# Autodesk Inventor assembly: DriveTrainPlateMecanum2017-18BackUp
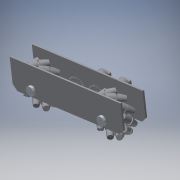
[picture p0: Inventor's stored thumbnail of the model, 180x180]
Saved by Autodesk Inventor 2017 (Build 210142000, 142)
## iProperties
Created: 2017-09-16
Part Number: DriveTrainPlateMecanum2017-18BackUp
Document SubType Name: Assembly
Designer: User
Author: User
## Documents named in this file (8)
- C:\Robotics\CAD\2017-18_CAD\DriveTrainMecanumDemo1.iam
- C:\Robotics\CAD\2017-18_CAD\MecanumDriveTrainPlate17-18.ipt
- C:\Robotics\CAD\2017-18_CAD\LeftDriveTrainMecanum2017-18.iam
- C:\Robotics\CAD\COTSParts\Motors\Andymark 2964  NeveRest 40 Motor.ipt
- C:\Robotics\CAD\2017-18_CAD\MecanumDriveTrainPlate17-18-NoMotor.ipt
- C:\Robotics\CAD\COTSParts\Tetrix\tetrix-motor-mounts-1.snapshot.1\Tetrex 2pc motor mount.ipt
- C:\Robotics\CAD\COTSParts\Actobotics\615 parts\615114.ipt
- C:\Robotics\CAD\COTSParts\Actobotics\545 parts\545576.ipt
## Components (12 placed, 7 different names)
1. LeftDriveTrainMecanum2017-18:1 [sub-assembly] — Mate:5, Mate:9, Mate:11, Mate:12
2. LeftDriveTrainMecanum2017-18:2 [sub-assembly] — Mate:6, Mate:7, Mate:10, Mate:13, Flush:3
3. MecanumDriveTrainPlate17-18:2 — Mate:5, Mate:6, Mate:7, Mate:9, Mate:12, Insert:1, Insert:2, Insert:3, Insert:4
4. Andymark 2964  NeveRest 40 Motor:1 — Mate:15, Flush:2, Mate:17
5. Andymark 2964  NeveRest 40 Motor:2 — Mate:14, Flush:1, Mate:16
6. MecanumDriveTrainPlate17-18-NoMotor:1 — Mate:10, Mate:11, Mate:13
7. Tetrex 2pc motor mount:1 — Insert:1, Insert:2, Mate:15, Flush:2
8. Tetrex 2pc motor mount:2 — Insert:3, Insert:4, Mate:14, Flush:1
9. 615114:1 — Mate:16, Flush:3, Flush:4, Insert:7, Insert:8
10. 615114:2 — Mate:17, Flush:4, Insert:5, Insert:6
11. 545576:1 — Insert:7, Insert:8
12. 545576:2 — Insert:5, Insert:6
## Relationships (24: Mate 12, Insert 8, Flush 4)
- Mate:5: LeftDriveTrainMecanum2017-18:1 ↔ MecanumDriveTrainPlate17-18:2
- Mate:6: LeftDriveTrainMecanum2017-18:2 ↔ MecanumDriveTrainPlate17-18:2
- Mate:7: LeftDriveTrainMecanum2017-18:2 ↔ MecanumDriveTrainPlate17-18:2
- Mate:9: LeftDriveTrainMecanum2017-18:1 ↔ MecanumDriveTrainPlate17-18:2
- Mate:10: LeftDriveTrainMecanum2017-18:2 ↔ MecanumDriveTrainPlate17-18-NoMotor:1
- Mate:11: LeftDriveTrainMecanum2017-18:1 ↔ MecanumDriveTrainPlate17-18-NoMotor:1
- Mate:12: LeftDriveTrainMecanum2017-18:1 ↔ MecanumDriveTrainPlate17-18:2
- Mate:13: LeftDriveTrainMecanum2017-18:2 ↔ MecanumDriveTrainPlate17-18-NoMotor:1
- Insert:1: MecanumDriveTrainPlate17-18:2 ↔ Tetrex 2pc motor mount:1
- Insert:2: MecanumDriveTrainPlate17-18:2 ↔ Tetrex 2pc motor mount:1
- Insert:3: MecanumDriveTrainPlate17-18:2 ↔ Tetrex 2pc motor mount:2
- Insert:4: MecanumDriveTrainPlate17-18:2 ↔ Tetrex 2pc motor mount:2
- Mate:14: Andymark 2964  NeveRest 40 Motor:2 ↔ Tetrex 2pc motor mount:2
- Mate:15: Andymark 2964  NeveRest 40 Motor:1 ↔ Tetrex 2pc motor mount:1
- Flush:1: Andymark 2964  NeveRest 40 Motor:2 ↔ Tetrex 2pc motor mount:2
- Flush:2: Andymark 2964  NeveRest 40 Motor:1 ↔ Tetrex 2pc motor mount:1
- Mate:16: Andymark 2964  NeveRest 40 Motor:2 ↔ 615114:1
- Flush:3: LeftDriveTrainMecanum2017-18:2 ↔ 615114:1
- Mate:17: Andymark 2964  NeveRest 40 Motor:1 ↔ 615114:2
- Flush:4: 615114:1 ↔ 615114:2
- Insert:5: 615114:2 ↔ 545576:2
- Insert:6: 615114:2 ↔ 545576:2
- Insert:7: 615114:1 ↔ 545576:1
- Insert:8: 615114:1 ↔ 545576:1
